# Autodesk Inventor assembly: FullWheel
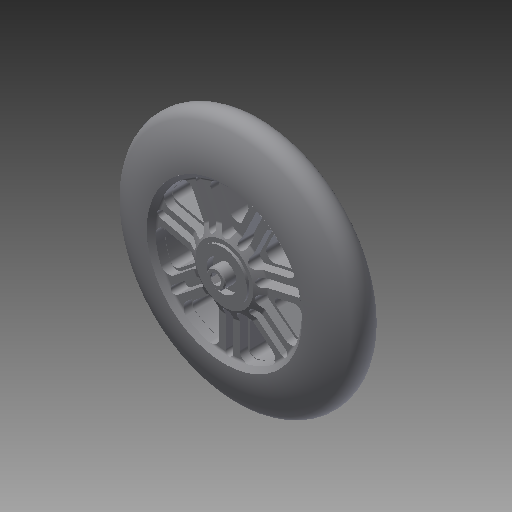
[picture p0: Inventor's stored thumbnail of the model, 512x512]
Saved by Autodesk Inventor 2019 (Build 230136000, 136)
## iProperties
Created: 2019-09-28
Part Number: FullWheel
Document SubType Name: Assembly
Designer: james
Author: james
## Documents named in this file (4)
- F:\JimsDesign\Jims2020FTC\FullWheel.iam
- F:\JimsDesign\Library\ServoCity\595626 assembly.iam
- F:\JimsDesign\Library\ServoCity\595630 assembly.iam
- F:\JimsDesign\Library\ServoCity\545578 assembly STEP File.iam
## Components (3 placed, 3 different names)
1. 595626 assembly:1 [sub-assembly] — Mate:1, Mate:2
2. 595630 assembly:1 [sub-assembly] — Mate:1, Mate:2, Mate:3, Mate:4, Mate:5
3. 545578 assembly STEP File:1 [sub-assembly] — Mate:3, Mate:4, Mate:5
## Relationships (5: Mate 5)
- Mate:1: 595626 assembly:1 ↔ 595630 assembly:1
- Mate:2: 595626 assembly:1 ↔ 595630 assembly:1
- Mate:3: 595630 assembly:1 ↔ 545578 assembly STEP File:1
- Mate:4: 595630 assembly:1 ↔ 545578 assembly STEP File:1
- Mate:5: 595630 assembly:1 ↔ 545578 assembly STEP File:1
